# Autodesk Inventor assembly: Application_openUC2_Discovery_Lightsheet
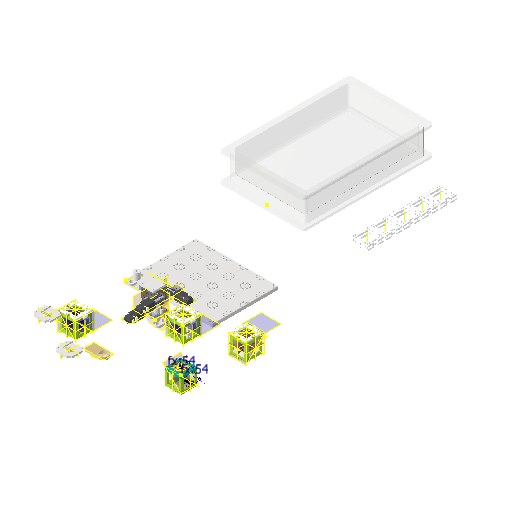
[picture p0: Inventor's stored thumbnail of the model, 512x512]
Saved by Autodesk Inventor 2025.1 (Build 291241020, 241B)
## iProperties
Created: 2022-07-25
Part Number: Application_openUC2_Discovery_Lightsheet
Document SubType Name: Assembly
Designer: diederichbenedict
Mass: 3654.94 g
Surface Area: 11054.2 cm^2
Volume: 3595.99 cm^3
Density: 1.01639 g/cm^3
Author: diederichbenedict
## Documents named in this file (8)
- C:\Users\diederichbenedict\Dropbox\Dokumente\Promotion\PROJECTS\openUC2-CAD\INVENTOR\Application_openUC2_Discovery_Lightsheet.iam
- C:\Users\diederichbenedict\Dropbox\Dokumente\Promotion\PROJECTS\openUC2-CAD\INVENTOR\10_Base_puzzle_v3.ipt
- C:\Users\diederichbenedict\Dropbox\Dokumente\Promotion\PROJECTS\openUC2-CAD\INVENTOR\00_Really_Useful_Box_4l_DinA4_body.ipt
- C:\Users\diederichbenedict\Dropbox\Dokumente\Promotion\PROJECTS\openUC2-CAD\INVENTOR\Assembly_Cube_FluorescenceFilterSlider.iam
- C:\Users\diederichbenedict\Dropbox\Dokumente\Promotion\PROJECTS\openUC2-CAD\INVENTOR\Assembly_XYZ_Stage_Micrometer_ontop_lightsheet.iam
- C:\Users\diederichbenedict\Dropbox\Dokumente\Promotion\PROJECTS\openUC2-CAD\INVENTOR\00_Baseplate_Lightsheet.ipt
- C:\Users\diederichbenedict\Dropbox\Dokumente\Promotion\PROJECTS\openUC2-CAD\INVENTOR\Assembly_Cube_Lightsheet_Sample_v3.iam
- C:\Users\diederichbenedict\Dropbox\Dokumente\Promotion\PROJECTS\openUC2-CAD\INVENTOR\Assembly_Cube_Lens_holder_CylindricalLens.iam
## Components (16 placed, 7 different names)
1. 00_Really_Useful_Box_4l_DinA4_body:1 — Passend:12
2. Assembly_Cube_FluorescenceFilterSlider:1 [sub-assembly]
3. Assembly_XYZ_Stage_Micrometer_ontop_lightsheet:1 [sub-assembly]
4. 00_Baseplate_Lightsheet:1
5. Assembly_Cube_Lightsheet_Sample_v3:1 [sub-assembly]
6. Assembly_Cube_Lens_holder_CylindricalLens:1 [sub-assembly]
7. 10_Base_puzzle_v3:1
8. 10_Base_puzzle_v3:2
9. 10_Base_puzzle_v3:3
10. 10_Base_puzzle_v3:4
11. 10_Base_puzzle_v3:5
12. 10_Base_puzzle_v3:6
13. 10_Base_puzzle_v3:7
14. 10_Base_puzzle_v3:8
15. 10_Base_puzzle_v3:9
16. 10_Base_puzzle_v3:10
## Component patterns: (10 elements, first: 10_Base_puzzle_v3:1)
## Relationships (1: Mate 1)
- Passend:12 [Mate]: 00_Really_Useful_Box_4l_DinA4_body:1
